# Autodesk Inventor assembly: Toughbox+Nano+All+Shafts+v2-2
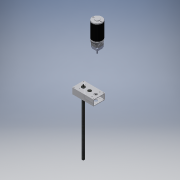
[picture p0: Inventor's stored thumbnail of the model, 180x180]
Saved by Autodesk Inventor 2016 (Build 200138000, 138)
## iProperties
Created: 2015-02-02
Part Number: Toughbox+Nano+All+Shafts+v2-2
Description: STEP AP203
Document SubType Name: Assembly
Designer: gus
Mass: 2193.65 g
Surface Area: 1474.64 cm^2
Volume: 577.261 cm^3
Density: 3.8001 g/cm^3
User Status: NEED!
Sending System: SolidWorks 2014
Preprocessor: SwSTEP 2.0
Title: Toughbox Nano All Shafts.STEP
Revision Number: ANY
## Documents named in this file (10)
- \\Mac\Home\Desktop\1510-stronghold-CAD-master\roller wheels\toughbox micro\Toughbox+Nano+All+Shafts+v2-2.iam
- \\Mac\Home\Desktop\1510-stronghold-CAD-master\roller wheels\toughbox micro\Toughbox Nano no Output Shaft.iam
- \\Mac\Home\Desktop\1510-stronghold-CAD-master\roller wheels\toughbox micro\500-e-klip_smart.ipt
- \\Mac\Home\Desktop\1510-stronghold-CAD-master\roller wheels\toughbox micro\TB Hex Output Shaft.ipt
- \\Mac\Home\Desktop\1510-stronghold-CAD-master\roller wheels\toughbox micro\CIM motor-1.ipt
- \\Mac\Home\Downloads\217-2820-STEP.iam
- \\Mac\Home\Downloads\217-2893.20121205.ipt
- \\Mac\Home\Downloads\217-4018-STEP-20140806.ipt
- \\Mac\Home\Desktop\1510-stronghold-CAD-master\roller wheels\cim vp\217-2816.20121205.ipt
- \\Mac\Home\Desktop\1510-stronghold-CAD-master\roller wheels\cim vp\vp bag motor\217-2625-002 Rev1.ipt
## Components (9 placed, 9 different names)
1. Toughbox Nano no Output Shaft_1 [sub-assembly] — Mate:12, Mate:13
2. 500-e-klip_smart_2
3. TB Hex Output Shaft_3
4. CIM motor-1_4 — Mate:1, Mate:2, Mate:3, Mate:6
5. 217-2820-STEP:1 [sub-assembly] — Flush:1, Mate:4
6. 217-2893.20121205:1 — Mate:11, Flush:3, Mate:13
7. 217-4018-STEP-20140806:1 — Mate:1, Mate:2, Mate:3, Mate:5, Mate:7
8. 217-2816.20121205:1 — Flush:1, Mate:4, Mate:5, Mate:6, Mate:7, Mate:8, Flush:2, Mate:9
9. 217-2625-002 Rev1:1 — Mate:8, Flush:2, Mate:9, Mate:11, Flush:3, Mate:12
## Relationships (15: Mate 12, Flush 3)
- Mate:1: CIM motor-1_4 ↔ 217-4018-STEP-20140806:1
- Mate:2: CIM motor-1_4 ↔ 217-4018-STEP-20140806:1
- Mate:3: CIM motor-1_4 ↔ 217-4018-STEP-20140806:1
- Flush:1: 217-2820-STEP:1 ↔ 217-2816.20121205:1
- Mate:4: 217-2820-STEP:1 ↔ 217-2816.20121205:1
- Mate:5: 217-4018-STEP-20140806:1 ↔ 217-2816.20121205:1
- Mate:6: CIM motor-1_4 ↔ 217-2816.20121205:1
- Mate:7: 217-4018-STEP-20140806:1 ↔ 217-2816.20121205:1
- Mate:8: 217-2816.20121205:1 ↔ 217-2625-002 Rev1:1
- Flush:2: 217-2816.20121205:1 ↔ 217-2625-002 Rev1:1
- Mate:9: 217-2816.20121205:1 ↔ 217-2625-002 Rev1:1
- Mate:11: 217-2893.20121205:1 ↔ 217-2625-002 Rev1:1
- Flush:3: 217-2893.20121205:1 ↔ 217-2625-002 Rev1:1
- Mate:12: Toughbox Nano no Output Shaft_1 ↔ 217-2625-002 Rev1:1
- Mate:13: Toughbox Nano no Output Shaft_1 ↔ 217-2893.20121205:1
